# Autodesk Inventor assembly: boxassem
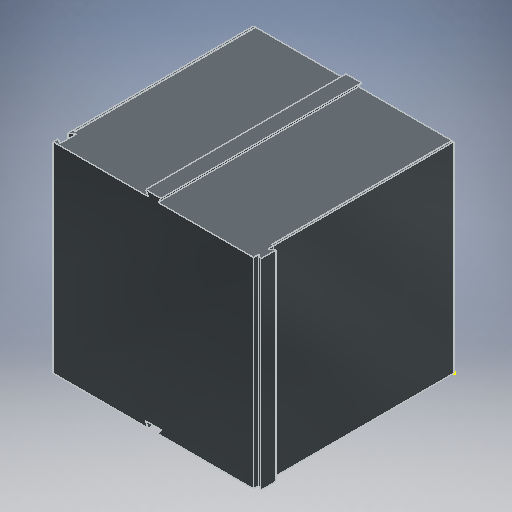
[picture p0: Inventor's stored thumbnail of the model, 512x512]
Saved by Autodesk Inventor 2025.2 (Build 292293000, 293)
## iProperties
Created: 2025-02-25
Part Number: boxassem
Document SubType Name: Assembly
Designer: email
Author: email
## Documents named in this file (3)
- C:\Shared\alex-bartella-schoolwork\4b03\dr3\V1\boxassem.iam
- C:\Shared\alex-bartella-schoolwork\4b03\dr3\V1\mainframe.ipt
- C:\Shared\alex-bartella-schoolwork\4b03\dr3\V1\side.ipt
## Components (3 placed, 2 different names)
1. mainframe:1 — Mate:7, Mate:8, Flush:1, Mate:9, Mate:10, Flush:2
2. side:1 — Mate:7, Mate:8, Flush:1
3. side:2 — Mate:9, Mate:10, Flush:2
## Relationships (6: Mate 4, Flush 2)
- Mate:7 (0.1 mm): mainframe:1 ↔ side:1
- Mate:8 (0.1 mm): mainframe:1 ↔ side:1
- Flush:1: mainframe:1 ↔ side:1
- Mate:9 (0.1 mm): mainframe:1 ↔ side:2
- Mate:10 (0.1 mm): mainframe:1 ↔ side:2
- Flush:2: mainframe:1 ↔ side:2
